# Autodesk Inventor assembly: elevation_assembly
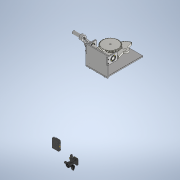
[picture p0: Inventor's stored thumbnail of the model, 180x180]
Saved by Autodesk Inventor 2020 (Build 240168000, 168)
## iProperties
Created: 2020-05-17
Part Number: elevation_assembly
Document SubType Name: Assembly
Designer: Hesekiel
Author: Hesekiel
## Documents named in this file (9)
- C:\Users\Hesekiel\Desktop\Equatorial-Mount-MUM\Mechanika\Mechanizm elewacji Filip\CAD\elevation_assembly.iam
- C:\Users\Hesekiel\Desktop\Equatorial-Mount-MUM\Mechanika\Mechanizm elewacji Filip\CAD\worm_gear.iam
- C:\Users\Hesekiel\Desktop\Equatorial-Mount-MUM\Mechanika\Mechanizm elewacji Filip\CAD\rack_and_pinion.iam
- C:\Users\Hesekiel\Desktop\Equatorial-Mount-MUM\Mechanika\Mechanizm elewacji Filip\CAD\wał_uzębienia.ipt
- C:\Users\Hesekiel\Desktop\Equatorial-Mount-MUM\Mechanika\Mechanizm elewacji Filip\CAD\M6x6_DIN914.ipt
- C:\Users\Hesekiel\Desktop\Equatorial-Mount-MUM\Mechanika\Mechanizm elewacji Filip\CAD\płyta_bazowa_elewacji.iam
- C:\Users\Hesekiel\Desktop\Equatorial-Mount-MUM\Mechanika\Mechanizm elewacji Filip\CAD\SKF 16006\16006.iam
- C:\Users\Hesekiel\Desktop\Equatorial-Mount-MUM\Mechanika\Mechanizm elewacji Filip\CAD\manfrotto-quick-release-plate\Manfrotto_501_PL_assem_01.iam
- C:\Users\Hesekiel\Desktop\Equatorial-Mount-MUM\Mechanika\Mechanizm elewacji Filip\CAD\manfrotto-494rc2-tripod-head.snapshot.1\Manfrotto 494RC2 - Tripod Head\Manfrotto - 494RC2 Head Assy.iam
## Components (10 placed, 8 different names)
1. worm_gear:1 [sub-assembly] — Mate:1, Mate:2, Rotational:4, Angle:1, Rotational:5
2. rack_and_pinion:1 [sub-assembly] — Mate:3, Mate:4
3. wał_uzębienia:1 — Mate:1, Mate:2, Rotational:4, Rigid:1, Mate:3, Mate:4, Rigid:5
4. M6x6_DIN914:1 — Rigid:1
5. M6x6_DIN914:2 — Rigid:5
6. płyta_bazowa_elewacji:1 [sub-assembly] — Mate:5, Rigid:3, Mate:6, Rigid:4
7. 16006:1 [sub-assembly] — Mate:5, Rigid:3, Rotational:5
8. 16006:2 [sub-assembly] — Mate:6, Rigid:4
9. Manfrotto_501_PL_assem_01:1 [sub-assembly]
10. Manfrotto - 494RC2 Head Assy:1 [sub-assembly]
## Relationships (13: Mate 6, WeldJoint 4, RevoluteJoint 2, Angle 1)
- Mate:1: worm_gear:1 ↔ wał_uzębienia:1
- Mate:2: worm_gear:1 ↔ wał_uzębienia:1
- Rotational:4 [RevoluteJoint]: worm_gear:1 ↔ wał_uzębienia:1
- Rigid:1 [WeldJoint]: wał_uzębienia:1 ↔ M6x6_DIN914:1
- Mate:3: rack_and_pinion:1 ↔ wał_uzębienia:1
- Mate:4: rack_and_pinion:1 ↔ wał_uzębienia:1
- Angle:1 (0 deg): worm_gear:1
- Mate:5: płyta_bazowa_elewacji:1 ↔ 16006:1
- Rigid:3 [WeldJoint]: płyta_bazowa_elewacji:1 ↔ 16006:1
- Mate:6: płyta_bazowa_elewacji:1 ↔ 16006:2
- Rigid:4 [WeldJoint]: płyta_bazowa_elewacji:1 ↔ 16006:2
- Rotational:5 [RevoluteJoint]: worm_gear:1 ↔ 16006:1
- Rigid:5 [WeldJoint]: wał_uzębienia:1 ↔ M6x6_DIN914:2
